# Autodesk Inventor assembly: motor
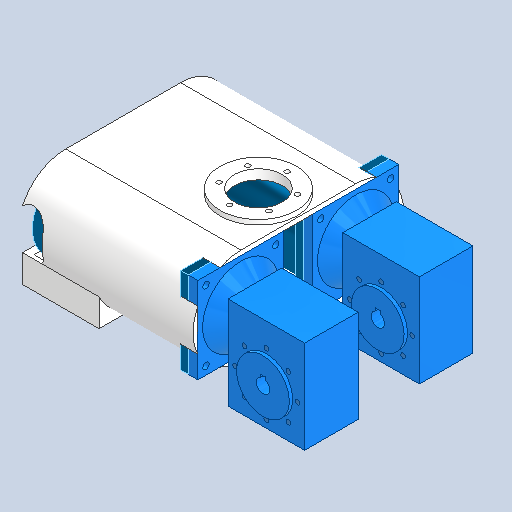
[picture p0: Inventor's stored thumbnail of the model, 512x512]
Saved by Autodesk Inventor 2025.3 (Build 293356030, 356C)
## iProperties
Created: 2025-09-06
Part Number: motor
Document SubType Name: Assembly
Designer: MSI
Author: MSI
## Documents named in this file (3)
- C:\Users\MSI\Desktop\Project\11. 로봇팔\Robot Arm Model\Robot_Arm_6_v1\motor.iam
- C:\Users\MSI\Desktop\Project\11. 로봇팔\Robot Arm Model\Robot_Arm_6_v1\NMRV30_motor.iam
- C:\Users\MSI\Desktop\Project\11. 로봇팔\Robot Arm Model\Robot_Arm_6_v1\motor_holder_1.ipt
## Components (3 placed, 2 different names)
1. NMRV30_motor:1 [sub-assembly] — 강체:1
2. NMRV30_motor:2 [sub-assembly] — 강체:2
3. motor_holder_1:1 — 강체:1, 강체:2
## Relationships (2: WeldJoint 2)
- 강체:1 [WeldJoint]: NMRV30_motor:1 ↔ motor_holder_1:1
- 강체:2 [WeldJoint]: NMRV30_motor:2 ↔ motor_holder_1:1
